# Autodesk Inventor assembly: MX-106T_with_Horn
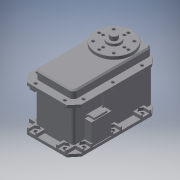
[picture p0: Inventor's stored thumbnail of the model, 180x180]
Saved by Autodesk Inventor 2016 (Build 200138000, 138)
## iProperties
Created: 2015-05-09
Part Number: MX-106T_with_Horn
Document SubType Name: Assembly
Designer: bitbots
Author: bitbots
## Documents named in this file (3)
- Z:\NICU\NICO_CAD_master\motors\Mx106\MX-106T_with_Horn.iam
- Z:\NICU\NICO_CAD_master\motors\Mx106\MX-106T.ipt
- Z:\NICU\NICO_CAD_master\motors\HN05-N101_(mx64)\HN05-N101.ipt
## Components (2 placed, 2 different names)
1. MX-106T:1 — Rotational:1
2. HN05-N101:1 — Rotational:1
## Relationships (1: RevoluteJoint 1)
- Rotational:1 [RevoluteJoint] (-7 mm): MX-106T:1 ↔ HN05-N101:1
